# Autodesk Inventor assembly: Assembly_Cube_Kinematic_Mirrormount_30x30_45_v3_aaa
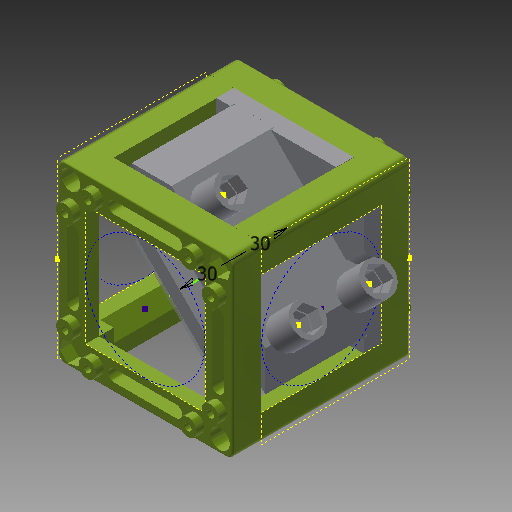
[picture p0: Inventor's stored thumbnail of the model, 512x512]
Saved by Autodesk Inventor 2019 (Build 230136000, 136)
## iProperties
Created: 2019-07-23
Part Number: Assembly_Cube_Kinematic_Mirrormount_30x30_45_v3_aaa
Document SubType Name: Assembly
Designer: marsikovabarbora
Mass: 52.0937 g
Surface Area: 280.4 cm^2
Volume: 41.3754 cm^3
Density: 1.25905 g/cm^3
Author: marsikovabarbora
## Documents named in this file (7)
- C:\Users\marsikovabarbora\Dropbox\UC2\02_CAD\INVENTOR\uc2_v3\Assembly_Cube_Kinematic_Mirrormount_30x30_45_v3.iam
- C:\Users\marsikovabarbora\Dropbox\UC2\02_CAD\INVENTOR\uc2_v3\Assembly_Cube_empty_IM_v3.iam
- C:\Users\marsikovabarbora\Dropbox\UC2\02_CAD\INVENTOR\uc2_v3\00_BallMagnets_5mm_single.ipt
- C:\Users\marsikovabarbora\Dropbox\UC2\02_CAD\INVENTOR\uc2_v3\20_Cube_Insert_Kinematic_Mirrormount_45_Plate.ipt
- C:\Users\marsikovabarbora\Dropbox\UC2\02_CAD\INVENTOR\uc2_v3\Assembly_Insert_Kinematic_Mirrormount_45_base.iam
- C:\Users\marsikovabarbora\Dropbox\UC2\02_CAD\INVENTOR\uc2_v3\openSIMv3\BAK\DIN 912 - M3 x 0,5 x 12 x 10,75.ipt
- C:\Users\marsikovabarbora\Dropbox\UC2\02_CAD\INVENTOR\uc2_v3\00_Mirror_30x30.ipt
## Components (9 placed, 6 different names)
1. Assembly_Cube_empty_IM_v3:1 [sub-assembly] — Mate:1, Mate:2, Mate:3, Passend:15, Fluchtend:10, Fluchtend:11
2. Assembly_Insert_Kinematic_Mirrormount_45_base:1 [sub-assembly] — Passend:13, Passend:14, Fluchtend:9, Passend:15, Fluchtend:10, Fluchtend:11, Winkel:1, Tangential:1, Winkel:2, Fluchtend:12
3. 00_BallMagnets_5mm_single:1 — Mate:8
4. 00_BallMagnets_5mm_single:2 — Mate:7
5. 00_BallMagnets_5mm_single:3 — Mate:6, Tangential:1
6. 20_Cube_Insert_Kinematic_Mirrormount_45_Plate:1 — Mate:6, Mate:7, Mate:8, Winkel:1, Winkel:2, Fluchtend:12, Passend:16, Fluchtend:13, Fluchtend:14
7. DIN 912 - ersetzt durch DIN EN ISO 4762 M3 x 12:1 — Passend:14, Fluchtend:8, Fluchtend:9
8. DIN 912 - ersetzt durch DIN EN ISO 4762 M3 x 12:2 — Passend:13, Fluchtend:8
9. 00_Mirror_30x30:1 — Passend:16, Fluchtend:13, Fluchtend:14
## Relationships (20: Mate 10, Flush 7, Angle 2, Tangent 1)
- Mate:1: Assembly_Cube_empty_IM_v3:1
- Mate:2: Assembly_Cube_empty_IM_v3:1
- Mate:3: Assembly_Cube_empty_IM_v3:1
- Mate:6: 00_BallMagnets_5mm_single:3 ↔ 20_Cube_Insert_Kinematic_Mirrormount_45_Plate:1
- Mate:7: 00_BallMagnets_5mm_single:2 ↔ 20_Cube_Insert_Kinematic_Mirrormount_45_Plate:1
- Mate:8: 00_BallMagnets_5mm_single:1 ↔ 20_Cube_Insert_Kinematic_Mirrormount_45_Plate:1
- Passend:13 [Mate]: Assembly_Insert_Kinematic_Mirrormount_45_base:1 ↔ DIN 912 - ersetzt durch DIN EN ISO 4762 M3 x 12:2
- Passend:14 [Mate]: Assembly_Insert_Kinematic_Mirrormount_45_base:1 ↔ DIN 912 - ersetzt durch DIN EN ISO 4762 M3 x 12:1
- Fluchtend:8 [Flush]: DIN 912 - ersetzt durch DIN EN ISO 4762 M3 x 12:1 ↔ DIN 912 - ersetzt durch DIN EN ISO 4762 M3 x 12:2
- Fluchtend:9 [Flush]: Assembly_Insert_Kinematic_Mirrormount_45_base:1 ↔ DIN 912 - ersetzt durch DIN EN ISO 4762 M3 x 12:1
- Passend:15 [Mate]: Assembly_Cube_empty_IM_v3:1 ↔ Assembly_Insert_Kinematic_Mirrormount_45_base:1
- Fluchtend:10 [Flush]: Assembly_Cube_empty_IM_v3:1 ↔ Assembly_Insert_Kinematic_Mirrormount_45_base:1
- Fluchtend:11 [Flush]: Assembly_Cube_empty_IM_v3:1 ↔ Assembly_Insert_Kinematic_Mirrormount_45_base:1
- Winkel:1 [Angle] (0 deg): Assembly_Insert_Kinematic_Mirrormount_45_base:1 ↔ 20_Cube_Insert_Kinematic_Mirrormount_45_Plate:1
- Tangential:1: Assembly_Insert_Kinematic_Mirrormount_45_base:1 ↔ 00_BallMagnets_5mm_single:3
- Winkel:2 [Angle] (180 deg): Assembly_Insert_Kinematic_Mirrormount_45_base:1 ↔ 20_Cube_Insert_Kinematic_Mirrormount_45_Plate:1
- Fluchtend:12 [Flush] (-2 mm): Assembly_Insert_Kinematic_Mirrormount_45_base:1 ↔ 20_Cube_Insert_Kinematic_Mirrormount_45_Plate:1
- Passend:16 [Mate]: 20_Cube_Insert_Kinematic_Mirrormount_45_Plate:1 ↔ 00_Mirror_30x30:1
- Fluchtend:13 [Flush]: 20_Cube_Insert_Kinematic_Mirrormount_45_Plate:1 ↔ 00_Mirror_30x30:1
- Fluchtend:14 [Flush] (5 mm): 20_Cube_Insert_Kinematic_Mirrormount_45_Plate:1 ↔ 00_Mirror_30x30:1
